# Autodesk Inventor assembly: Poste de travail_MIR
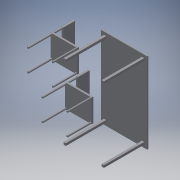
[picture p0: Inventor's stored thumbnail of the model, 180x180]
Saved by Autodesk Inventor 2016 SP1 (Build 200210100, 210)
## iProperties
Created: 2016-10-04
Part Number: Poste de travail_MIR
Material: Générique
Document SubType Name: Assembly
Designer: dimercur
Author: dimercur
EcartPiedChaise: 100,000 mm
ChaiseAvancée: 300,000 mm
ChaiseReculée: 550,000 mm
## Documents named in this file (3)
- D:\Users\dimercur\Documents\SVN\projets-gei\Salle 22-24\Poste de travail_MIR.iam
- D:\Users\dimercur\Documents\SVN\projets-gei\Salle 22-24\Chaise_MIR.ipt
- D:\Users\dimercur\Documents\SVN\projets-gei\Salle 22-24\Table_MIR.ipt
## Components (3 placed, 2 different names)
1. Chaise_MIR:1 — Placage:3, Placage:2, Affleurement:1
2. Chaise_MIR:2 — Placage:4, Affleurement:2, Placage:1
3. Table_MIR:1 — Placage:4, Placage:3, Placage:2, Affleurement:2, Affleurement:1, Placage:1
## Relationships (6: Mate 4, Flush 2)
- Placage:4 [Mate] (550 mm): Chaise_MIR:2 ↔ Table_MIR:1
- Placage:3 [Mate] (300 mm): Chaise_MIR:1 ↔ Table_MIR:1
- Placage:2 [Mate] (100 mm): Chaise_MIR:1 ↔ Table_MIR:1
- Affleurement:2 [Flush]: Chaise_MIR:2 ↔ Table_MIR:1
- Affleurement:1 [Flush]: Chaise_MIR:1 ↔ Table_MIR:1
- Placage:1 [Mate] (100 mm): Chaise_MIR:2 ↔ Table_MIR:1
